# Autodesk Inventor assembly: cajas_V2
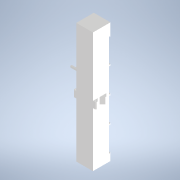
[picture p0: Inventor's stored thumbnail of the model, 180x180]
Saved by Autodesk Inventor 2020.3 (Build 243373000, 373)
## iProperties
Created: 2021-03-07
Part Number: cajas_V2
Document SubType Name: Assembly
Designer: juanp
Author: juanp
## Documents named in this file (3)
- C:\Users\juanp\Desktop\Robocol\Nuevo EVA\V1\Cajas\cajas_V2.iam
- C:\Users\juanp\Desktop\Robocol\Nuevo EVA\V1\Cajas\cajas_V2.ipt
- C:\Users\juanp\Desktop\Robocol\Nuevo EVA\V1\Cajas\Adaptador SG90.ipt
## Components (2 placed, 2 different names)
1. cajas_V2:1 — Mate:1, Mate:3, Mate:4
2. Adaptador SG90:1 — Mate:1, Mate:3, Mate:4
## Relationships (3: Mate 3)
- Mate:1: cajas_V2:1 ↔ Adaptador SG90:1
- Mate:3: cajas_V2:1 ↔ Adaptador SG90:1
- Mate:4: cajas_V2:1 ↔ Adaptador SG90:1
